# Autodesk Inventor assembly: Truc_Z
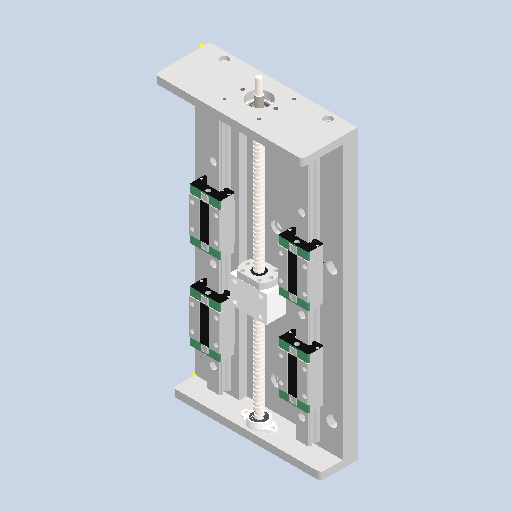
[picture p0: Inventor's stored thumbnail of the model, 512x512]
Saved by Autodesk Inventor 2023 (Build 270158000, 158)
## iProperties
Created: 2025-04-17
Part Number: Truc_Z
Document SubType Name: Assembly
Designer: huyqu
Author: huyqu
## Documents named in this file (6)
- E:\TAI LIEU\Final_Project\DONE\CoCauTrucZ\Truc_Z.iam
- E:\TAI LIEU\Final_Project\DONE\CoCauTrucZ\khung_doc.ipt
- E:\TAI LIEU\Final_Project\DONE\CoCauTrucZ\Nap_tren.ipt
- E:\TAI LIEU\Final_Project\DONE\CoCauTrucZ\Nap_duoi.ipt
- E:\TAI LIEU\Final_Project\DONE\CoCauTrucZ\Ray_Truot.iam
- E:\TAI LIEU\Final_Project\DONE\CoCauTrucZ\vitme_aogoi\vitme_aogoi.iam
## Components (6 placed, 5 different names)
1. khung_doc:1 — Mate:1, Mate:2, Mate:3, Mate:4, Mate:5, Mate:6, Mate:7, Mate:8, Mate:9, Mate:10, Mate:11, Mate:12
2. Nap_tren:1 — Mate:1, Mate:2, Mate:3
3. Nap_duoi:1 — Mate:4, Mate:5, Mate:6, Mate:13, Mate:14
4. Ray_Truot:1 [sub-assembly] — Mate:7, Mate:8, Mate:9
5. Ray_Truot:2 [sub-assembly] — Mate:10, Mate:11, Mate:12
6. vitme_aogoi:1 [sub-assembly] — Mate:13, Mate:14
## Relationships (14: Mate 14)
- Mate:1: khung_doc:1 ↔ Nap_tren:1
- Mate:2: khung_doc:1 ↔ Nap_tren:1
- Mate:3: khung_doc:1 ↔ Nap_tren:1
- Mate:4: khung_doc:1 ↔ Nap_duoi:1
- Mate:5: khung_doc:1 ↔ Nap_duoi:1
- Mate:6: khung_doc:1 ↔ Nap_duoi:1
- Mate:7: khung_doc:1 ↔ Ray_Truot:1
- Mate:8: khung_doc:1 ↔ Ray_Truot:1
- Mate:9: khung_doc:1 ↔ Ray_Truot:1
- Mate:10: khung_doc:1 ↔ Ray_Truot:2
- Mate:11: khung_doc:1 ↔ Ray_Truot:2
- Mate:12: khung_doc:1 ↔ Ray_Truot:2
- Mate:13: Nap_duoi:1 ↔ vitme_aogoi:1
- Mate:14: Nap_duoi:1 ↔ vitme_aogoi:1
